# Autodesk Inventor assembly: Vertical Lift
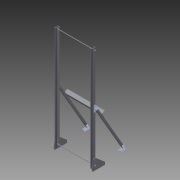
[picture p0: Inventor's stored thumbnail of the model, 180x180]
Saved by Autodesk Inventor 2015 SP1 (Build 190203100, 203)
## iProperties
Created: 2015-01-13
Part Number: Vertical Lift
Document SubType Name: Assembly
Designer: Jarod
Author: Jarod
## Documents named in this file (11)
- C:\Users\Jarod\Documents\Westview\Robotics\FRC\2015\CAD\Robot\Vertical Lift\Vertical Lift.iam
- C:\Users\Jarod\Documents\Westview\Robotics\FRC\2015\CAD\Robot\Vertical Lift\garage door 2in rail.ipt
- C:\Users\Jarod\Documents\Westview\Robotics\FRC\2015\CAD\Robot\Vertical Lift\rail aligner.ipt
- C:\Users\Jarod\Documents\Westview\Robotics\FRC\2015\CAD\Robot\Vertical Lift\garage door 2in rail_MIR.ipt
- C:\Users\Jarod\Documents\Westview\Robotics\FRC\2015\CAD\Robot\Vertical Lift\rail mounting bracket.ipt
- C:\Users\Jarod\Documents\Westview\Robotics\FRC\2015\CAD\Robot\Vertical Lift\0.375 axle.ipt
- C:\Users\Jarod\Documents\Westview\Robotics\FRC\2015\CAD\Robot\Vertical Lift\Imported Components\0.375 shaft collar\0.375 shaft collar.ipt
- C:\Users\Jarod\Documents\Westview\Robotics\FRC\2015\CAD\Robot\Vertical Lift\Imported Components\Versaframe 30deg gusset\Versaframe 30deg gusset.ipt
- C:\Users\Jarod\Documents\Westview\Robotics\FRC\2015\CAD\Robot\Vertical Lift\Imported Components\Versaframe 60deg gusset\Versaframe 60deg gusset.ipt
- C:\Users\Jarod\Documents\Westview\Robotics\FRC\2015\CAD\Robot\Vertical Lift\1x1 support.ipt
- C:\Users\Jarod\Documents\Westview\Robotics\FRC\2015\CAD\Robot\Vertical Lift\2x2 angle support.ipt
## Components (23 placed, 10 different names)
1. garage door 2in rail:1 — Mate:44, Flush:5, Mate:45, Flush:7, Mate:48, Flush:8, Mate:90, Mate:91, Mate:108, Mate:110, Mate:111, Mate:112, Flush:20
2. garage door 2in rail_MIR:1 — Mate:46, Mate:47, Flush:6, Flush:7, Mate:48, Mate:92, Flush:9, Mate:93, Flush:11, Mate:98, Mate:104, Mate:106, Mate:113, Mate:114, Flush:21
3. rail aligner:1 — Mate:46, Mate:47, Flush:6
4. rail aligner:2 — Mate:44, Flush:5, Mate:45
5. rail mounting bracket:1 — Flush:8, Mate:90, Mate:91, Mate:102
6. rail mounting bracket:2 — Mate:92, Flush:9, Mate:93, Mate:97, Flush:10, Mate:100
7. 0.375 axle:1 — Mate:97, Flush:10, Mate:99, Mate:101
8. 0.375 axle:2 — Flush:11, Mate:98, Mate:103, Mate:105, Mate:107, Mate:109
9. 0.375 shaft collar:1 — Mate:99, Mate:100
10. 0.375 shaft collar:2 — Mate:101, Mate:102
11. 0.375 shaft collar:3 — Mate:103, Mate:104
12. 0.375 shaft collar:4 — Mate:105, Mate:106
13. 0.375 shaft collar:5 — Mate:107, Mate:108
14. 0.375 shaft collar:6 — Mate:109, Mate:110
15. Versaframe 30deg gusset:1 — Mate:111, Mate:112, Mate:115, Flush:12, Mate:124, Mate:130
16. Versaframe 30deg gusset:2 — Mate:113, Mate:114, Mate:116, Flush:13, Mate:127, Mate:131
17. Versaframe 60deg gusset:1 — Mate:117, Flush:14, Flush:18, Flush:20, Mate:121, Mate:122
18. Versaframe 60deg gusset:2 — Mate:118, Flush:15, Flush:18
19. Versaframe 60deg gusset:3 — Mate:119, Flush:16, Flush:19, Mate:125, Mate:126
20. Versaframe 60deg gusset:4 — Mate:120, Flush:17, Flush:19, Flush:21
21. 1x1 support:1 — Mate:115, Flush:12, Mate:117, Flush:14, Mate:118, Flush:15, Mate:121, Mate:122, Mate:124, Mate:129, Flush:22, Flush:23, Mate:130
22. 1x1 support:2 — Mate:116, Flush:13, Mate:119, Flush:16, Mate:120, Flush:17, Mate:125, Mate:126, Mate:127, Mate:131
23. 2x2 angle support:1 — Mate:129, Flush:22, Flush:23
## Relationships (61: Mate 42, Flush 19)
- Mate:44: garage door 2in rail:1 ↔ rail aligner:2
- Flush:5: garage door 2in rail:1 ↔ rail aligner:2
- Mate:45: garage door 2in rail:1 ↔ rail aligner:2
- Mate:46: garage door 2in rail_MIR:1 ↔ rail aligner:1
- Mate:47: garage door 2in rail_MIR:1 ↔ rail aligner:1
- Flush:6: garage door 2in rail_MIR:1 ↔ rail aligner:1
- Flush:7: garage door 2in rail:1 ↔ garage door 2in rail_MIR:1
- Mate:48 (-552.45 mm): garage door 2in rail:1 ↔ garage door 2in rail_MIR:1
- Flush:8 (-38.1 mm): garage door 2in rail:1 ↔ rail mounting bracket:1
- Mate:90: garage door 2in rail:1 ↔ rail mounting bracket:1
- Mate:91: garage door 2in rail:1 ↔ rail mounting bracket:1
- Mate:92: garage door 2in rail_MIR:1 ↔ rail mounting bracket:2
- Flush:9 (-38.1 mm): garage door 2in rail_MIR:1 ↔ rail mounting bracket:2
- Mate:93: garage door 2in rail_MIR:1 ↔ rail mounting bracket:2
- Mate:97: rail mounting bracket:2 ↔ 0.375 axle:1
- Flush:10 (-22.225 mm): rail mounting bracket:2 ↔ 0.375 axle:1
- Flush:11 (-28.575 mm): garage door 2in rail_MIR:1 ↔ 0.375 axle:2
- Mate:98: garage door 2in rail_MIR:1 ↔ 0.375 axle:2
- Mate:99: 0.375 axle:1 ↔ 0.375 shaft collar:1
- Mate:100: rail mounting bracket:2 ↔ 0.375 shaft collar:1
- Mate:101: 0.375 axle:1 ↔ 0.375 shaft collar:2
- Mate:102: rail mounting bracket:1 ↔ 0.375 shaft collar:2
- Mate:103: 0.375 axle:2 ↔ 0.375 shaft collar:3
- Mate:104: garage door 2in rail_MIR:1 ↔ 0.375 shaft collar:3
- Mate:105: 0.375 axle:2 ↔ 0.375 shaft collar:4
- Mate:106: garage door 2in rail_MIR:1 ↔ 0.375 shaft collar:4
- Mate:107: 0.375 axle:2 ↔ 0.375 shaft collar:5
- Mate:108: garage door 2in rail:1 ↔ 0.375 shaft collar:5
- Mate:109: 0.375 axle:2 ↔ 0.375 shaft collar:6
- Mate:110: garage door 2in rail:1 ↔ 0.375 shaft collar:6
- Mate:111 (-25.4 mm): garage door 2in rail:1 ↔ Versaframe 30deg gusset:1
- Mate:112: garage door 2in rail:1 ↔ Versaframe 30deg gusset:1
- Mate:113: garage door 2in rail_MIR:1 ↔ Versaframe 30deg gusset:2
- Mate:114 (-25.4 mm): garage door 2in rail_MIR:1 ↔ Versaframe 30deg gusset:2
- Mate:115: Versaframe 30deg gusset:1 ↔ 1x1 support:1
- Flush:12: Versaframe 30deg gusset:1 ↔ 1x1 support:1
- Mate:116: Versaframe 30deg gusset:2 ↔ 1x1 support:2
- Flush:13: Versaframe 30deg gusset:2 ↔ 1x1 support:2
- Mate:117: Versaframe 60deg gusset:1 ↔ 1x1 support:1
- Flush:14: Versaframe 60deg gusset:1 ↔ 1x1 support:1
- Mate:118: Versaframe 60deg gusset:2 ↔ 1x1 support:1
- Flush:15: Versaframe 60deg gusset:2 ↔ 1x1 support:1
- Mate:119: Versaframe 60deg gusset:3 ↔ 1x1 support:2
- Flush:16: Versaframe 60deg gusset:3 ↔ 1x1 support:2
- Mate:120: Versaframe 60deg gusset:4 ↔ 1x1 support:2
- Flush:17: Versaframe 60deg gusset:4 ↔ 1x1 support:2
- Flush:18: Versaframe 60deg gusset:1 ↔ Versaframe 60deg gusset:2
- Flush:19: Versaframe 60deg gusset:3 ↔ Versaframe 60deg gusset:4
- Flush:20: garage door 2in rail:1 ↔ Versaframe 60deg gusset:1
- Flush:21: garage door 2in rail_MIR:1 ↔ Versaframe 60deg gusset:4
- Mate:121 (0.127 mm): Versaframe 60deg gusset:1 ↔ 1x1 support:1
- Mate:122 (0.127 mm): Versaframe 60deg gusset:1 ↔ 1x1 support:1
- Mate:124 (0.127 mm): Versaframe 30deg gusset:1 ↔ 1x1 support:1
- Mate:125 (0.127 mm): Versaframe 60deg gusset:3 ↔ 1x1 support:2
- Mate:126 (0.127 mm): Versaframe 60deg gusset:3 ↔ 1x1 support:2
- Mate:127 (0.127 mm): Versaframe 30deg gusset:2 ↔ 1x1 support:2
- Mate:129: 1x1 support:1 ↔ 2x2 angle support:1
- Flush:22: 1x1 support:1 ↔ 2x2 angle support:1
- Flush:23 (622.3 mm): 1x1 support:1 ↔ 2x2 angle support:1
- Mate:130 (0.127 mm): Versaframe 30deg gusset:1 ↔ 1x1 support:1
- Mate:131 (0.127 mm): Versaframe 30deg gusset:2 ↔ 1x1 support:2
